# Autodesk Inventor assembly: цепь_MIR4
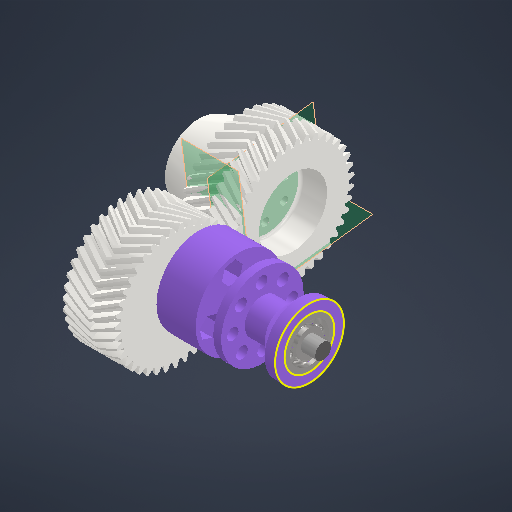
[picture p0: Inventor's stored thumbnail of the model, 512x512]
Saved by Autodesk Inventor 2025 (Build 290162000, 162)
## iProperties
Created: 2024-07-09
Part Number: цепь_MIR4
Document SubType Name: Assembly
Designer: Phantom
Author: Phantom
## Documents named in this file (6)
- C:\Users\Phantom\Desktop\Phantom16950\цепь_MIR4.iam
- C:\Users\Phantom\Desktop\Phantom16950\втулка для подш 2 часть_MIR6.ipt
- C:\Users\Phantom\Desktop\Phantom16950\втулка для подш_MIR6.ipt
- C:\Users\Phantom\Desktop\Phantom16950\Деталь_64_MIR6.ipt
- C:\Users\Phantom\Desktop\Phantom16950\BS 290 SKF - SKF 626-RZ_MIR6.ipt
- C:\Users\Phantom\Desktop\Phantom16950\цепь\Мастер проектирования\Цилиндрическое зубчатое зацепление4_MIR.iam
## Components (6 placed, 5 different names)
1. втулка для подш 2 часть_MIR6:1 — Совмещение:16, Совмещение:23, Совмещение:20
2. втулка для подш_MIR6:1 — Совмещение:16, Совмещение:17, Совмещение:25
3. Деталь_64_MIR6:1 — Совмещение:23, Совмещение:17, Совмещение:21, Совмещение:19
4. BS 290 SKF - SKF 626-RZ_MIR6:1 — Совмещение:21, Совмещение:20
5. BS 290 SKF - SKF 626-RZ_MIR6:2 — Совмещение:19, Совмещение:27
6. Цилиндрическое зубчатое зацепление4_MIR:1 [sub-assembly] — Совмещение:27, Совмещение:25
## Relationships (8: Mate 8)
- Совмещение:16 [Mate]: втулка для подш 2 часть_MIR6:1 ↔ втулка для подш_MIR6:1
- Совмещение:23 [Mate]: втулка для подш 2 часть_MIR6:1 ↔ Деталь_64_MIR6:1
- Совмещение:17 [Mate]: втулка для подш_MIR6:1 ↔ Деталь_64_MIR6:1
- Совмещение:21 [Mate]: Деталь_64_MIR6:1 ↔ BS 290 SKF - SKF 626-RZ_MIR6:1
- Совмещение:20 [Mate]: втулка для подш 2 часть_MIR6:1 ↔ BS 290 SKF - SKF 626-RZ_MIR6:1
- Совмещение:19 [Mate]: Деталь_64_MIR6:1 ↔ BS 290 SKF - SKF 626-RZ_MIR6:2
- Совмещение:27 [Mate]: BS 290 SKF - SKF 626-RZ_MIR6:2 ↔ Цилиндрическое зубчатое зацепление4_MIR:1
- Совмещение:25 [Mate]: втулка для подш_MIR6:1 ↔ Цилиндрическое зубчатое зацепление4_MIR:1
